# Autodesk Inventor assembly: 1-RIE_CS44 Connetor-0.040Shielded
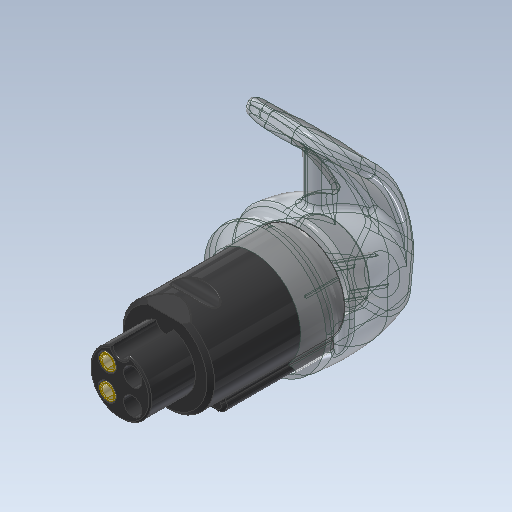
[picture p0: Inventor's stored thumbnail of the model, 512x512]
Saved by Autodesk Inventor 2020 (Build 240168000, 168)
## iProperties
Created: 2014-10-23
Part Number: 1-RIE_CS44 Connetor-0.040Shielded
Document SubType Name: Assembly
Designer: Mark Neilson
Mass: 0.072881 g
Surface Area: 2.75303 cm^2
Volume: 0.0625862 cm^3
Density: 1.16449 g/cm^3
Author: Mark Neilson
## Documents named in this file (4)
- C:\Users\alex.lynch\Nextcloud\Documents\UCSD OpenSpeech\CAD\DJB parametric CAD files\200226\1-RIE_CS44 Connetor-0.040Shielded.iam
- C:\Users\alex.lynch\Nextcloud\Documents\UCSD OpenSpeech\CAD\DJB parametric CAD files\200226\1-95a4180.ipt
- C:\Users\alex.lynch\Nextcloud\Documents\UCSD OpenSpeech\CAD\DJB parametric CAD files\200226\1-95a4191.ipt
- C:\Users\alex.lynch\Nextcloud\Documents\UCSD OpenSpeech\CAD\DJB parametric CAD files\200226\9-RIE_009P-024.ipt
## Components (4 placed, 3 different names)
1. 1-95a4180.ipt:1 — Insert:1, Insert:2
2. 1-95a4191.ipt:2
3. 9-RIE_009P-024.ipt:3 — Insert:2
4. 9-RIE_009P-024.ipt:4 — Insert:1
## Relationships (2: Insert 2)
- Insert:1: 1-95a4180.ipt:1 ↔ 9-RIE_009P-024.ipt:4
- Insert:2: 1-95a4180.ipt:1 ↔ 9-RIE_009P-024.ipt:3
